# Autodesk Inventor assembly: Pancake_Timing Assy_Lever Shaft
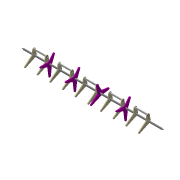
[picture p0: Inventor's stored thumbnail of the model, 180x180]
Saved by Autodesk Inventor 2018.1 (Build 221171000, 171)
## iProperties
Created: 2019-02-11
Part Number: Pancake_Timing Assy_Lever Shaft
Document SubType Name: Assembly
Designer: James
Author: James
## Documents named in this file (8)
- C:\Users\admin\Desktop\Ball-Machine\Pancake Sort\Pancake_Timing Assy_Lever Shaft.iam
- C:\Users\admin\Desktop\Ball-Machine\Timing Gate\Timing_Lever.ipt
- C:\Users\admin\Desktop\Ball-Machine\Pancake Sort\BS 3673 - 6mm External Circlip.ipt
- C:\Users\admin\Desktop\Ball-Machine\Timing Gate\M3 x 0.5mm Zinc Plated Steel Washer.ipt
- C:\Users\admin\Desktop\Ball-Machine\Timing Gate\Socket Button Head - (A2) - M3 x 10.ipt
- C:\Users\admin\Desktop\Ball-Machine\Pancake Sort\Pancake_Lever Shaft.ipt
- C:\Users\admin\Desktop\Ball-Machine\Pancake Sort\Pancake_Lever Weight.ipt
- C:\Users\admin\Desktop\Ball-Machine\Pancake Sort\Pancake_Switch Lever 2.ipt
## Components (107 placed, 7 different names)
1. Pancake_Lever Shaft:1 — Mate:45, Flush:18, Mate:46, Mate:47, Mate:48, Mate:49, Mate:56, Mate:62, Mate:63, Mate:64, Mate:65, Mate:66, Mate:68, Mate:69, Mate:70, Mate:71, Flush:23, Flush:24, Flush:25, Flush:26, Mate:84, Mate:86
2. Pancake_Switch Lever 2:5 — Mate:68, Flush:23
3. Pancake_Switch Lever 2:6 — Mate:69, Flush:24
4. Pancake_Switch Lever 2:7 — Mate:70, Flush:26
5. Pancake_Switch Lever 2:8 — Mate:71, Flush:25
6. BS 3673 - 6mm External Circlip:2 — Flush:10, Angle:2, Mate:47, Mate:48, Flush:19, Mate:85
7. BS 3673 - 6mm External Circlip:1 — Flush:10, Mate:46, Mate:49, Flush:19, Angle:3
8. BS 3673 - 6mm External Circlip:3 — Mate:61, Flush:20
9. BS 3673 - 6mm External Circlip:4
10. BS 3673 - 6mm External Circlip:5
11. BS 3673 - 6mm External Circlip:6
12. BS 3673 - 6mm External Circlip:7
13. BS 3673 - 6mm External Circlip:8
14. BS 3673 - 6mm External Circlip:9
15. BS 3673 - 6mm External Circlip:10
16. BS 3673 - 6mm External Circlip:11
17. BS 3673 - 6mm External Circlip:12
18. BS 3673 - 6mm External Circlip:13
19. BS 3673 - 6mm External Circlip:14
20. BS 3673 - 6mm External Circlip:15
21. BS 3673 - 6mm External Circlip:16
22. BS 3673 - 6mm External Circlip:17
23. BS 3673 - 6mm External Circlip:18
24. BS 3673 - 6mm External Circlip:19
25. BS 3673 - 6mm External Circlip:20
26. Socket Button Head - (A2) - M3 x 10:1 — Mate:15, Mate:16
27. M3 x 0.5mm Zinc Plated Steel Washer:1 — Mate:13, Mate:14, Mate:15
28. Timing_Lever:1 — Mate:7, Mate:8, Mate:13, Mate:14, Mate:16, Mate:45, Flush:18, Angle:4
29. Pancake_Lever Weight:1 — Mate:7, Mate:8, Mate:59, Mate:60
30. Socket Button Head - (A2) - M3 x 10:2 — Mate:52, Mate:54
31. M3 x 0.5mm Zinc Plated Steel Washer:2 — Mate:54, Mate:55
32. Timing_Lever:7 — Mate:56, Mate:59, Mate:52, Mate:55, Mate:60, Mate:61, Flush:22
33. Socket Button Head - (A2) - M3 x 10:3
34. M3 x 0.5mm Zinc Plated Steel Washer:3
35. Timing_Lever:2
36. Pancake_Lever Weight:2
37. Socket Button Head - (A2) - M3 x 10:4
38. M3 x 0.5mm Zinc Plated Steel Washer:4
39. Timing_Lever:8
40. Socket Button Head - (A2) - M3 x 10:5
41. M3 x 0.5mm Zinc Plated Steel Washer:5
42. Timing_Lever:3
43. Pancake_Lever Weight:3
44. Socket Button Head - (A2) - M3 x 10:6
45. M3 x 0.5mm Zinc Plated Steel Washer:6
46. Timing_Lever:9
47. Socket Button Head - (A2) - M3 x 10:7
48. M3 x 0.5mm Zinc Plated Steel Washer:7
49. Timing_Lever:4
50. Pancake_Lever Weight:4
51. Socket Button Head - (A2) - M3 x 10:8
52. M3 x 0.5mm Zinc Plated Steel Washer:8
53. Timing_Lever:10
54. Socket Button Head - (A2) - M3 x 10:9
55. M3 x 0.5mm Zinc Plated Steel Washer:9
56. Timing_Lever:5
57. Pancake_Lever Weight:5
58. Socket Button Head - (A2) - M3 x 10:10
59. M3 x 0.5mm Zinc Plated Steel Washer:10
60. Timing_Lever:11
61. BS 3673 - 6mm External Circlip:22 — Mate:62, Mate:65, Flush:20, Flush:21, Mate:67
62. Pancake_Switch Lever 2:1 — Mate:66, Mate:67, Flush:22
63. BS 3673 - 6mm External Circlip:21 — Mate:63, Mate:64, Flush:21
64. BS 3673 - 6mm External Circlip:23
65. Pancake_Switch Lever 2:2
66. BS 3673 - 6mm External Circlip:24
67. BS 3673 - 6mm External Circlip:25
68. Pancake_Switch Lever 2:3
69. BS 3673 - 6mm External Circlip:26
70. BS 3673 - 6mm External Circlip:27
71. Pancake_Switch Lever 2:4
72. BS 3673 - 6mm External Circlip:28
73. Timing_Lever:12 — Mate:84, Mate:85
74. Pancake_Lever Weight:6
75. M3 x 0.5mm Zinc Plated Steel Washer:11
76. Socket Button Head - (A2) - M3 x 10:11
77. M3 x 0.5mm Zinc Plated Steel Washer:12
78. Socket Button Head - (A2) - M3 x 10:12
79. Timing_Lever:13 — Mate:86
80. Timing_Lever:14
81. Pancake_Lever Weight:7
82. M3 x 0.5mm Zinc Plated Steel Washer:13
83. Socket Button Head - (A2) - M3 x 10:13
84. M3 x 0.5mm Zinc Plated Steel Washer:14
85. Socket Button Head - (A2) - M3 x 10:14
86. Timing_Lever:15
87. Timing_Lever:16
88. Pancake_Lever Weight:8
89. M3 x 0.5mm Zinc Plated Steel Washer:15
90. Socket Button Head - (A2) - M3 x 10:15
91. M3 x 0.5mm Zinc Plated Steel Washer:16
92. Socket Button Head - (A2) - M3 x 10:16
93. Timing_Lever:17
94. Timing_Lever:18
95. Pancake_Lever Weight:9
96. M3 x 0.5mm Zinc Plated Steel Washer:17
97. Socket Button Head - (A2) - M3 x 10:17
98. M3 x 0.5mm Zinc Plated Steel Washer:18
99. Socket Button Head - (A2) - M3 x 10:18
100. Timing_Lever:19
101. Timing_Lever:20
102. Pancake_Lever Weight:10
103. M3 x 0.5mm Zinc Plated Steel Washer:19
104. Socket Button Head - (A2) - M3 x 10:19
105. M3 x 0.5mm Zinc Plated Steel Washer:20
106. Socket Button Head - (A2) - M3 x 10:20
107. Timing_Lever:21
## Component patterns: (10 elements, first: BS 3673 - 6mm External Circlip:2 + BS 3673 - 6mm External Circlip:1), (5 elements, first: Socket Button Head - (A2) - M3 x 10:1 + M3 x 0.5mm Zinc Plated Steel Washer:1 + Timing_Lever:1 + Pancake_Lever Weight:1 + Socket Button Head - (A2) - M3 x 10:2 + M3 x 0.5mm Zinc Plated Steel Washer:2 + Timing_Lever:7), (4 elements, first: BS 3673 - 6mm External Circlip:22 + Pancake_Switch Lever 2:1 + BS 3673 - 6mm External Circlip:21), (5 elements, first: Timing_Lever:12 + Pancake_Lever Weight:6 + M3 x 0.5mm Zinc Plated Steel Washer:11 + Socket Button Head - (A2) - M3 x 10:11 + M3 x 0.5mm Zinc Plated Steel Washer:12 + Socket Button Head - (A2) - M3 x 10:12 + Timing_Lever:13)
## Relationships (63: Mate 44, Flush 16, Angle 3)
- [Flush]: Pancake_Lever Shaft:1
- Mate:7: Timing_Lever:1 ↔ Pancake_Lever Weight:1
- Mate:8: Timing_Lever:1 ↔ Pancake_Lever Weight:1
- Flush:10: BS 3673 - 6mm External Circlip:2 ↔ BS 3673 - 6mm External Circlip:1
- Angle:2 (180 deg): BS 3673 - 6mm External Circlip:2
- Mate:13: M3 x 0.5mm Zinc Plated Steel Washer:1 ↔ Timing_Lever:1
- Mate:14: M3 x 0.5mm Zinc Plated Steel Washer:1 ↔ Timing_Lever:1
- Mate:15: Socket Button Head - (A2) - M3 x 10:1 ↔ M3 x 0.5mm Zinc Plated Steel Washer:1
- Mate:16: Socket Button Head - (A2) - M3 x 10:1 ↔ Timing_Lever:1
- Flush:11 (-58 mm)
- Flush:12 (-5 mm)
- Flush:13 (30 mm)
- [Flush]: Pancake_Lever Shaft:1
- [Flush]: Pancake_Lever Shaft:1
- Mate:45: Pancake_Lever Shaft:1 ↔ Timing_Lever:1
- Flush:18: Pancake_Lever Shaft:1 ↔ Timing_Lever:1
- Mate:46: Pancake_Lever Shaft:1 ↔ BS 3673 - 6mm External Circlip:1
- Mate:47: Pancake_Lever Shaft:1 ↔ BS 3673 - 6mm External Circlip:2
- Mate:48: Pancake_Lever Shaft:1 ↔ BS 3673 - 6mm External Circlip:2
- Mate:49: Pancake_Lever Shaft:1 ↔ BS 3673 - 6mm External Circlip:1
- Flush:19: BS 3673 - 6mm External Circlip:2 ↔ BS 3673 - 6mm External Circlip:1
- Angle:3 (0 deg): BS 3673 - 6mm External Circlip:1
- [Mate]: Socket Button Head - (A2) - M3 x 10:2 ↔ M3 x 0.5mm Zinc Plated Steel Washer:2
- Mate:52: Socket Button Head - (A2) - M3 x 10:2 ↔ Timing_Lever:7
- Mate:54: Socket Button Head - (A2) - M3 x 10:2 ↔ M3 x 0.5mm Zinc Plated Steel Washer:2
- Mate:55: M3 x 0.5mm Zinc Plated Steel Washer:2 ↔ Timing_Lever:7
- Mate:56: Pancake_Lever Shaft:1 ↔ Timing_Lever:7
- Mate:59: Pancake_Lever Weight:1 ↔ Timing_Lever:7
- Mate:60: Pancake_Lever Weight:1 ↔ Timing_Lever:7
- Mate:61: BS 3673 - 6mm External Circlip:3 ↔ Timing_Lever:7
- Angle:4 (7.5 deg): Timing_Lever:1
- Mate:62: Pancake_Lever Shaft:1 ↔ BS 3673 - 6mm External Circlip:22
- Mate:63: Pancake_Lever Shaft:1 ↔ BS 3673 - 6mm External Circlip:21
- Mate:64: Pancake_Lever Shaft:1 ↔ BS 3673 - 6mm External Circlip:21
- Mate:65: Pancake_Lever Shaft:1 ↔ BS 3673 - 6mm External Circlip:22
- Flush:20: BS 3673 - 6mm External Circlip:3 ↔ BS 3673 - 6mm External Circlip:22
- Flush:21: BS 3673 - 6mm External Circlip:22 ↔ BS 3673 - 6mm External Circlip:21
- Mate:66: Pancake_Lever Shaft:1 ↔ Pancake_Switch Lever 2:1
- Mate:67: BS 3673 - 6mm External Circlip:22 ↔ Pancake_Switch Lever 2:1
- Flush:22: Timing_Lever:7 ↔ Pancake_Switch Lever 2:1
- Mate:68: Pancake_Lever Shaft:1 ↔ Pancake_Switch Lever 2:5
- Mate:69: Pancake_Lever Shaft:1 ↔ Pancake_Switch Lever 2:6
- Mate:70: Pancake_Lever Shaft:1 ↔ Pancake_Switch Lever 2:7
- Mate:71: Pancake_Lever Shaft:1 ↔ Pancake_Switch Lever 2:8
- Flush:23: Pancake_Lever Shaft:1 ↔ Pancake_Switch Lever 2:5
- Flush:24: Pancake_Lever Shaft:1 ↔ Pancake_Switch Lever 2:6
- Flush:25: Pancake_Lever Shaft:1 ↔ Pancake_Switch Lever 2:8
- Flush:26: Pancake_Lever Shaft:1 ↔ Pancake_Switch Lever 2:7
- [Mate]: Timing_Lever:12 ↔ Pancake_Lever Weight:6
- [Mate]: Timing_Lever:12 ↔ Pancake_Lever Weight:6
- [Mate]: Timing_Lever:12 ↔ M3 x 0.5mm Zinc Plated Steel Washer:11
- [Mate]: Timing_Lever:12 ↔ M3 x 0.5mm Zinc Plated Steel Washer:11
- [Mate]: M3 x 0.5mm Zinc Plated Steel Washer:11 ↔ Socket Button Head - (A2) - M3 x 10:11
- [Mate]: Timing_Lever:12 ↔ Socket Button Head - (A2) - M3 x 10:11
- [Mate]: M3 x 0.5mm Zinc Plated Steel Washer:12 ↔ Socket Button Head - (A2) - M3 x 10:12
- [Mate]: Socket Button Head - (A2) - M3 x 10:12 ↔ Timing_Lever:13
- [Mate]: M3 x 0.5mm Zinc Plated Steel Washer:12 ↔ Socket Button Head - (A2) - M3 x 10:12
- [Mate]: M3 x 0.5mm Zinc Plated Steel Washer:12 ↔ Timing_Lever:13
- [Mate]: Pancake_Lever Weight:6 ↔ Timing_Lever:13
- [Mate]: Pancake_Lever Weight:6 ↔ Timing_Lever:13
- Mate:84: Pancake_Lever Shaft:1 ↔ Timing_Lever:12
- Mate:85: BS 3673 - 6mm External Circlip:2 ↔ Timing_Lever:12
- Mate:86: Pancake_Lever Shaft:1 ↔ Timing_Lever:13
## Named parameters: d204_d35 = 0 mm, d274_d20 = 0 mm, d275_d21 = 0 mm, d276_d204_d35 = 0 mm, d277_d205 = 0 mm, d278_d207 = 0 mm, d279_d208 = 0 mm, d280_d233 = 0 mm, d281_d234 = 0 mm, d282_d33 = 0 mm, d283_d34 = 0 mm, d284_d35 = 0 mm, d285_d36 = 0 mm
